# Autodesk Inventor assembly: Con_Vibraciones_Bancada
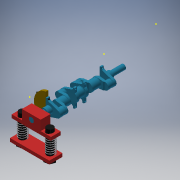
[picture p0: Inventor's stored thumbnail of the model, 180x180]
Saved by Autodesk Inventor 2019 (Build 230136000, 136)
## iProperties
Created: 2019-07-01
Part Number: Con_Vibraciones_Bancada
Document SubType Name: Assembly
Designer: Oscar Rojas
Author: Oscar Rojas
## Documents named in this file (8)
- E:\OSCAR\UNAL\6to SEMESTRE\Principios de dinámica\Proyectos\Proyecto 2\Mio\Con_Vibraciones_Bancada.iam
- E:\OSCAR\UNAL\6to SEMESTRE\Principios de dinámica\Proyectos\Proyecto 2\Mio\cigueñal.ipt
- E:\OSCAR\UNAL\6to SEMESTRE\Principios de dinámica\Proyectos\Proyecto 2\Mio\ContrapesoGrande1.ipt
- E:\OSCAR\UNAL\6to SEMESTRE\Principios de dinámica\Proyectos\Proyecto 2\Mio\Pasador.ipt
- E:\OSCAR\UNAL\6to SEMESTRE\Principios de dinámica\Proyectos\Proyecto 2\Mio\SuperiorBancada.ipt
- E:\OSCAR\UNAL\6to SEMESTRE\Principios de dinámica\Proyectos\Proyecto 2\Mio\Tornillo.ipt
- E:\OSCAR\UNAL\6to SEMESTRE\Principios de dinámica\Proyectos\Proyecto 2\Mio\BaseBancada.ipt
- E:\OSCAR\UNAL\6to SEMESTRE\Principios de dinámica\Proyectos\Proyecto 2\Mio\Resorte.ipt
## Components (10 placed, 7 different names)
1. cigueñal:1 — Rotational:1, Insert:3
2. ContrapesoGrande1:1 — Rotational:1, Insert:1, Insert:2
3. Pasador:1 — Insert:2
4. Pasador:2 — Insert:1
5. SuperiorBancada:1 — Insert:3, Rigid:1
6. Tornillo:1 — Insert:4
7. Tornillo:2 — Insert:5
8. BaseBancada:1 — Insert:4, Insert:5, Rigid:1
9. Resorte:1
10. Resorte:2
## Relationships (7: Insert 5, RevoluteJoint 1, WeldJoint 1)
- Rotational:1 [RevoluteJoint]: cigueñal:1 ↔ ContrapesoGrande1:1
- Insert:1 (-15 mm): ContrapesoGrande1:1 ↔ Pasador:2
- Insert:2 (-15 mm): ContrapesoGrande1:1 ↔ Pasador:1
- Insert:3 (-20 mm): cigueñal:1 ↔ SuperiorBancada:1
- Insert:4: Tornillo:1 ↔ BaseBancada:1
- Insert:5: Tornillo:2 ↔ BaseBancada:1
- Rigid:1 [WeldJoint] (10 mm): SuperiorBancada:1 ↔ BaseBancada:1
